# Autodesk Inventor assembly: ALOHA2_viperx
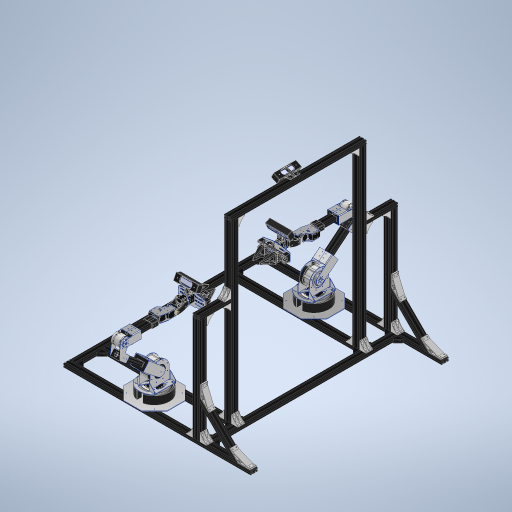
[picture p0: Inventor's stored thumbnail of the model, 512x512]
Saved by Autodesk Inventor 2024.3 (Build 283343010, 343A)
## iProperties
Created: 2025-08-13
Part Number: ALOHA2_viperx
Document SubType Name: Assembly
Designer: kshau
Author: kshau
## Documents named in this file (3)
- C:\Users\kshau\Documents\inventor\Create_ViperX\Create_ViperX_ALOHA\ILOHA_overall.iam
- C:\Users\kshau\Documents\inventor\Create_ViperX\Create_ViperX_ALOHA\ILOHA_Frame.iam
- C:\Users\kshau\Documents\inventor\Create_ViperX\Create_ViperX_ALOHA\ILOHA_Arm.iam
## Components (3 placed, 2 different names)
1. ILOHA_Frame:1 [sub-assembly] — メイト:1, フラッシュ:1, メイト:2, フラッシュ:4
2. ILOHA_Arm:1 [sub-assembly] — フラッシュ:2, フラッシュ:3, フラッシュ:4
3. ILOHA_Arm:2 [sub-assembly] — メイト:1, フラッシュ:1, メイト:2, フラッシュ:2, フラッシュ:3
## Relationships (6: Flush 4, Mate 2)
- メイト:1 [Mate]: ILOHA_Frame:1 ↔ ILOHA_Arm:2
- フラッシュ:1 [Flush] (-15 mm): ILOHA_Frame:1 ↔ ILOHA_Arm:2
- メイト:2 [Mate] (245 mm): ILOHA_Frame:1 ↔ ILOHA_Arm:2
- フラッシュ:2 [Flush]: ILOHA_Arm:1 ↔ ILOHA_Arm:2
- フラッシュ:3 [Flush]: ILOHA_Arm:1 ↔ ILOHA_Arm:2
- フラッシュ:4 [Flush] (-15 mm): ILOHA_Frame:1 ↔ ILOHA_Arm:1
